# Autodesk Inventor assembly: EChem_200 Cap
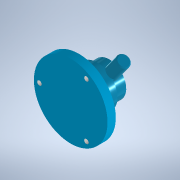
[picture p0: Inventor's stored thumbnail of the model, 180x180]
Saved by Autodesk Inventor 2021 (Build 250183000, 183)
## iProperties
Created: 2020-07-06
Part Number: EChem_200 Cap
Document SubType Name: Assembly
Designer: jgray
Author: jgray
## Documents named in this file (3)
- M:\Printed Electronics\Gas Sensors\Prototypes\Prototype II -Cartridge Reader V3\EChem_200 Cap.iam
- M:\Printed Electronics\Gas Sensors\Prototypes\Prototype II -Cartridge Reader V3\EChem _S200 Cap Top.ipt
- M:\Printed Electronics\Gas Sensors\Prototypes\Prototype II -Cartridge Reader V3\EChem _S200 Cap Base.ipt
## Components (2 placed, 2 different names)
1. EChem _S200 Cap Top:1 — Mate:1, Mate:2
2. EChem _S200 Cap Base:1 — Mate:1, Mate:2
## Relationships (2: Mate 2)
- Mate:1: EChem _S200 Cap Top:1 ↔ EChem _S200 Cap Base:1
- Mate:2: EChem _S200 Cap Top:1 ↔ EChem _S200 Cap Base:1
